# Autodesk Inventor assembly: Arm Assembly
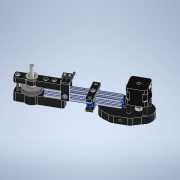
[picture p0: Inventor's stored thumbnail of the model, 180x180]
Saved by Autodesk Inventor 2022 (Build 260153000, 153)
## iProperties
Created: 2022-04-09
Part Number: Arm Assembly
Document SubType Name: Assembly
Designer: JK
Author: JK
## Documents named in this file (23)
- C:\Users\JK\Documents\Inventor\ScaraNema\SCARA-3DP\Parts\Arm\Arm Assembly.iam
- C:\Users\JK\Documents\Inventor\ScaraNema\SCARA-3DP\Parts\Shoulder\Platform.ipt
- C:\Users\JK\Documents\Inventor\ScaraNema\SCARA-3DP\Parts\Shoulder\MOTOR.ipt
- C:\Users\JK\Documents\Inventor\ScaraNema\SCARA-3DP\Parts\Shoulder\Motor spacer.ipt
- C:\Users\JK\Documents\Inventor\ScaraNema\SCARA-3DP\Parts\Shoulder\M3x35.ipt
- C:\Users\JK\Documents\Inventor\ScaraNema\SCARA-3DP\Parts\Shoulder\GT2 16 Pulley.ipt
- C:\Users\JK\Documents\Inventor\ScaraNema\SCARA-3DP\Parts\V-Slot 20x20\V-Slot 20x20x150.ipt
- C:\Users\JK\Documents\Inventor\ScaraNema\SCARA-3DP\Parts\V-Slot 20x20.ipt
- C:\Users\JK\Documents\Inventor\ScaraNema\SCARA-3DP\Parts\Shoulder\Belt tensor.ipt
- C:\Users\JK\Documents\Inventor\ScaraNema\SCARA-3DP\Parts\Shoulder\Idle pulley 16\GT2-16 Idle pulley.iam
- C:\Users\JK\Documents\Inventor\ScaraNema\SCARA-3DP\Parts\Shoulder\M3x25Socket Bolt.ipt
- C:\Users\JK\Documents\Inventor\ScaraNema\SCARA-3DP\Parts\Shoulder\M3Nut.ipt
- C:\Users\JK\Documents\Inventor\ScaraNema\SCARA-3DP\Parts\Shoulder\PernoM5x8Plano.ipt
- C:\Users\JK\Documents\Inventor\ScaraNema\SCARA-3DP\Parts\Shoulder\M5x20BoltFlatHead.ipt
- C:\Users\JK\Documents\Inventor\ScaraNema\SCARA-3DP\Parts\Shoulder\M5Nut.ipt
- C:\Users\JK\Documents\Inventor\ScaraNema\SCARA-3DP\Parts\Shoulder\M5x10.ipt
- C:\Users\JK\Documents\Inventor\ScaraNema\SCARA-3DP\Parts\Shoulder\TuercaTM5Perfil2020.ipt
- C:\Users\JK\Documents\Inventor\ScaraNema\SCARA-3DP\Parts\Elbow\Elbow assembly.iam
- C:\Users\JK\Documents\Inventor\ScaraNema\SCARA-3DP\Parts\endstopsupportarm.ipt
- C:\Users\JK\Documents\Inventor\ScaraNema\SCARA-3DP\Parts\PernoM5x8Plano.ipt
- C:\Users\JK\Documents\Inventor\ScaraNema\SCARA-3DP\Parts\25T0397-001.ipt
- C:\Users\JK\Documents\Inventor\ScaraNema\SCARA-3DP\Parts\Shoulder\M2bolt.ipt
- C:\Users\JK\Documents\Inventor\ScaraNema\SCARA-3DP\Parts\Shoulder\91828A111_18-8 Stainless Steel Hex Nut.ipt
## Components (38 placed, 20 different names)
1. Platform:1
2. MOTOR:1
3. GT2 16 Pulley:1
4. V-Slot 20x20x150:1 — Coincidencia:36, Nivelación:12, Coincidencia:37, Nivelación:13, Coincidencia:43
5. Belt tensor:1
6. GT2-16 Idle pulley:1 [sub-assembly]
7. GT2-16 Idle pulley:2 [sub-assembly]
8. M3x25Socket Bolt:1
9. M3x25Socket Bolt:2
10. M3Nut:1
11. M3Nut:2
12. PernoM5x8Plano:1
13. M5x20BoltFlatHead:1
14. M5x20BoltFlatHead:2
15. M5Nut:1
16. M5Nut:2
17. M5x10:1
18. M5x10:2
19. TuercaTM5Perfil2020:1
20. TuercaTM5Perfil2020:2
21. TuercaTM5Perfil2020:3
22. Elbow assembly:1 [sub-assembly] — Coincidencia:36, Nivelación:12, Coincidencia:37, Nivelación:14
23. endstopsupportarm:1 — Nivelación:13, Coincidencia:39, Coincidencia:40, Coincidencia:41, Coincidencia:42, Coincidencia:43, Nivelación:14, Coincidencia:44, Coincidencia:45, Coincidencia:46, Ángulo:9, Coincidencia:52
24. PernoM5x8Plano:2 — Coincidencia:39, Coincidencia:41
25. PernoM5x8Plano:3 — Coincidencia:40, Coincidencia:42
26. 25T0397-001:1 — Coincidencia:44, Coincidencia:45, Coincidencia:46, Coincidencia:47, Coincidencia:48, Coincidencia:49
27. M2bolt:1 — Coincidencia:47, Nivelación:15, Coincidencia:49, Coincidencia:50
28. M2bolt:2 — Coincidencia:48, Nivelación:15, Coincidencia:51
29. 91828A111_18-8 Stainless Steel Hex Nut:1 — Coincidencia:50, Ángulo:8, Nivelación:16, Coincidencia:52
30. 91828A111_18-8 Stainless Steel Hex Nut:2 — Coincidencia:51, Ángulo:8, Ángulo:9, Nivelación:16
31. Motor spacer:1
32. M3x35:1
33. M3x35:2
34. Motor spacer:2
35. M3x35:3
36. Motor spacer:3
37. M3x35:4
38. Motor spacer:4
## Component patterns: (4 elements, first: Motor spacer:1 + M3x35:1)
## Relationships (76: Mate 51, Flush 16, Angle 9)
- [Mate]: Platform:1 ↔ Motor spacer:1
- [Mate]: Platform:1 ↔ Motor spacer:1
- [Mate]: MOTOR:1 ↔ Motor spacer:1
- [Mate]: Motor spacer:1 ↔ M3x35:1
- [Mate]: Platform:1 ↔ M3x35:1
- [Mate]: MOTOR:1 ↔ GT2 16 Pulley:1
- [Flush] (-6.25 mm): Platform:1 ↔ GT2 16 Pulley:1
- [Angle] (90 deg): Platform:1 ↔ MOTOR:1
- [Mate]: Platform:1 ↔ MOTOR:1
- [Mate]: Platform:1 ↔ V-Slot 20x20x150:1
- [Flush] (-25 mm): Platform:1 ↔ V-Slot 20x20x150:1
- [Mate] (10 mm): MOTOR:1 ↔ V-Slot 20x20x150:1
- [Mate] (0.15 mm): V-Slot 20x20x150:1 ↔ Belt tensor:1
- [Mate] (0.15 mm): V-Slot 20x20x150:1 ↔ Belt tensor:1
- [Flush] (-50 mm): V-Slot 20x20x150:1 ↔ Belt tensor:1
- [Mate]: Belt tensor:1 ↔ GT2-16 Idle pulley:1
- [Mate]: Belt tensor:1 ↔ GT2-16 Idle pulley:2
- [Flush]: GT2-16 Idle pulley:1 ↔ GT2-16 Idle pulley:2
- [Mate] (4 mm): Belt tensor:1 ↔ GT2-16 Idle pulley:1
- [Mate]: Belt tensor:1 ↔ M3x25Socket Bolt:1
- [Mate]: Belt tensor:1 ↔ M3x25Socket Bolt:2
- [Mate]: Belt tensor:1 ↔ M3x25Socket Bolt:2
- [Flush]: M3x25Socket Bolt:1 ↔ M3x25Socket Bolt:2
- [Mate]: M3x25Socket Bolt:1 ↔ M3Nut:2
- [Angle] (0 deg): Belt tensor:1 ↔ M3Nut:2
- [Mate]: M3x25Socket Bolt:2 ↔ M3Nut:1
- [Angle] (0 deg): Belt tensor:1 ↔ M3Nut:1
- [Mate]: Belt tensor:1 ↔ M3Nut:1
- [Flush]: M3Nut:1 ↔ M3Nut:2
- [Mate]: Belt tensor:1 ↔ PernoM5x8Plano:1
- [Mate]: Belt tensor:1 ↔ PernoM5x8Plano:1
- [Mate]: Platform:1 ↔ M5x20BoltFlatHead:1
- [Mate]: Platform:1 ↔ M5x20BoltFlatHead:1
- [Mate]: Platform:1 ↔ M5x20BoltFlatHead:2
- [Flush]: M5x20BoltFlatHead:1 ↔ M5x20BoltFlatHead:2
- [Mate]: Platform:1 ↔ M5Nut:1
- [Mate]: Platform:1 ↔ M5Nut:2
- [Angle] (0 deg): MOTOR:1 ↔ M5Nut:2
- [Flush]: M5Nut:1 ↔ M5Nut:2
- [Mate]: Platform:1 ↔ M5Nut:1
- [Mate]: Platform:1 ↔ M5Nut:2
- [Mate]: Platform:1 ↔ M5x10:1
- [Mate]: Platform:1 ↔ M5x10:2
- [Mate]: M5x20BoltFlatHead:2 ↔ TuercaTM5Perfil2020:1
- [Mate]: M5x20BoltFlatHead:1 ↔ TuercaTM5Perfil2020:2
- [Flush]: TuercaTM5Perfil2020:1 ↔ TuercaTM5Perfil2020:2
- [Angle] (0 deg): Belt tensor:1 ↔ TuercaTM5Perfil2020:2
- [Angle] (0 deg): TuercaTM5Perfil2020:1 ↔ TuercaTM5Perfil2020:2
- [Flush]: M5x20BoltFlatHead:2 ↔ TuercaTM5Perfil2020:1
- [Flush]: TuercaTM5Perfil2020:1 ↔ TuercaTM5Perfil2020:2
- [Mate]: PernoM5x8Plano:1 ↔ TuercaTM5Perfil2020:3
- [Angle] (0 deg): Belt tensor:1 ↔ TuercaTM5Perfil2020:3
- [Mate] (0.6 mm): Belt tensor:1 ↔ TuercaTM5Perfil2020:3
- Coincidencia:36 [Mate]: V-Slot 20x20x150:1 ↔ Elbow assembly:1
- Nivelación:12 [Flush]: V-Slot 20x20x150:1 ↔ Elbow assembly:1
- Coincidencia:37 [Mate] (-40 mm): V-Slot 20x20x150:1 ↔ Elbow assembly:1
- Nivelación:13 [Flush]: V-Slot 20x20x150:1 ↔ endstopsupportarm:1
- Coincidencia:39 [Mate]: endstopsupportarm:1 ↔ PernoM5x8Plano:2
- Coincidencia:40 [Mate]: endstopsupportarm:1 ↔ PernoM5x8Plano:3
- Coincidencia:41 [Mate]: endstopsupportarm:1 ↔ PernoM5x8Plano:2
- Coincidencia:42 [Mate]: endstopsupportarm:1 ↔ PernoM5x8Plano:3
- Coincidencia:43 [Mate] (0.15 mm): V-Slot 20x20x150:1 ↔ endstopsupportarm:1
- Nivelación:14 [Flush] (-10 mm): Elbow assembly:1 ↔ endstopsupportarm:1
- Coincidencia:44 [Mate]: endstopsupportarm:1 ↔ 25T0397-001:1
- Coincidencia:45 [Mate]: endstopsupportarm:1 ↔ 25T0397-001:1
- Coincidencia:46 [Mate]: endstopsupportarm:1 ↔ 25T0397-001:1
- Coincidencia:47 [Mate]: 25T0397-001:1 ↔ M2bolt:1
- Coincidencia:48 [Mate]: 25T0397-001:1 ↔ M2bolt:2
- Nivelación:15 [Flush]: M2bolt:1 ↔ M2bolt:2
- Coincidencia:49 [Mate]: 25T0397-001:1 ↔ M2bolt:1
- Coincidencia:50 [Mate]: M2bolt:1 ↔ 91828A111_18-8 Stainless Steel Hex Nut:1
- Coincidencia:51 [Mate]: M2bolt:2 ↔ 91828A111_18-8 Stainless Steel Hex Nut:2
- Ángulo:8 [Angle] (0 deg): 91828A111_18-8 Stainless Steel Hex Nut:1 ↔ 91828A111_18-8 Stainless Steel Hex Nut:2
- Ángulo:9 [Angle] (0 deg): endstopsupportarm:1 ↔ 91828A111_18-8 Stainless Steel Hex Nut:2
- Nivelación:16 [Flush]: 91828A111_18-8 Stainless Steel Hex Nut:1 ↔ 91828A111_18-8 Stainless Steel Hex Nut:2
- Coincidencia:52 [Mate]: endstopsupportarm:1 ↔ 91828A111_18-8 Stainless Steel Hex Nut:1
## Named parameters: d11_d41 = 0 mm, d12_d42 = 0 mm, d13_d45 = 0 mm, d14_d46 = 0 mm, d15_d47 = 0 mm, d16_d48 = 90 deg, d17_d49 = 4, d19_d50 = 0 mm, d20_d51 = -6.25 mm, d21_d52 = 90 deg, d22_d53 = 0 mm, d23_d54 = 0 mm, d24_d55 = -25 mm
